# Autodesk Inventor assembly: Durometer_Assembly
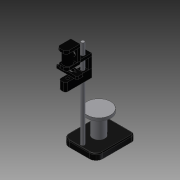
[picture p0: Inventor's stored thumbnail of the model, 180x180]
Saved by Autodesk Inventor 2015 (Build 190159000, 159)
## iProperties
Created: 2014-12-16
Part Number: Durometer_Assembly
Document SubType Name: Assembly
Designer: amarschn
Author: amarschn
## Documents named in this file (5)
- \\andrew.ad.cmu.edu\users\users7\amarschn\Documents\Durometer_Assembly\Durometer_Assembly.iam
- \\andrew.ad.cmu.edu\users\users7\amarschn\Documents\Durometer_Assembly\Durometer_Base.ipt
- \\andrew.ad.cmu.edu\users\users7\amarschn\Documents\Durometer_Assembly\Durometer_Slide_Shaft.ipt
- \\andrew.ad.cmu.edu\users\users7\amarschn\Documents\Durometer_Assembly\Durometer_Platform.ipt
- \\andrew.ad.cmu.edu\users\users7\amarschn\Documents\Durometer_Assembly\Durometer_Slide_Fixture.iam
## Components (4 placed, 4 different names)
1. Durometer_Base:1 — Insert:1, Flush:1, Mate:1
2. Durometer_Slide_Shaft:1 — Insert:1, Mate:2, Flush:2
3. Durometer_Platform:1 — Flush:1, Mate:1
4. Durometer_Slide_Fixture:1 [sub-assembly] — Mate:2, Flush:2
## Relationships (5: Flush 2, Mate 2, Insert 1)
- Insert:1: Durometer_Base:1 ↔ Durometer_Slide_Shaft:1
- Flush:1: Durometer_Base:1 ↔ Durometer_Platform:1
- Mate:1: Durometer_Base:1 ↔ Durometer_Platform:1
- Mate:2: Durometer_Slide_Shaft:1 ↔ Durometer_Slide_Fixture:1
- Flush:2 (50 mm): Durometer_Slide_Shaft:1 ↔ Durometer_Slide_Fixture:1
